# Autodesk Inventor assembly: populated-keyboard_cherrymx
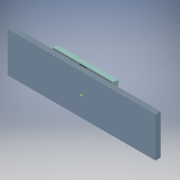
[picture p0: Inventor's stored thumbnail of the model, 180x180]
Saved by Autodesk Inventor 2018 (Build 220112000, 112)
## iProperties
Created: 2016-12-08
Part Number: populated-keyboard_cherrymx
Document SubType Name: Assembly
Designer: Cemra JC
Author: Cemra JC
## Documents named in this file (10)
- C:\Users\Jason Cemra\Documents\Logical Store\StenoToppers\stenotoppers\cherrymx\mockup-parts\populated-keyboard_cherrymx.iam
- C:\Users\Jason Cemra\Documents\Logical Store\StenoToppers\stenotoppers\cherrymx\mockup-parts\keyboard-mockup_cherrymx.iam
- C:\Users\Jason Cemra\Documents\Logical Store\StenoToppers\stenotoppers\cherrymx\mockup-parts\cherry-mx-switch\keyswitch_cherrymx.iam
- C:\Users\Jason Cemra\Documents\Logical Store\StenoToppers\stenotoppers\cherrymx\mockup-parts\spacebar-keycap_mockup_cherrymx.ipt
- C:\Users\Jason Cemra\Documents\Logical Store\StenoToppers\stenotoppers\cherrymx\stenotoppers\standard_cmx.ipt
- C:\Users\Jason Cemra\Documents\Logical Store\StenoToppers\stenotoppers\cherrymx\stenotoppers\smaller_cmx.ipt
- C:\Users\Jason Cemra\Documents\Logical Store\StenoToppers\stenotoppers\cherrymx\stenotoppers\larger_cmx.ipt
- C:\Users\Jason Cemra\Documents\Logical Store\StenoToppers\stenotoppers\cherrymx\stenotoppers\thumb_cmx.ipt
- J:\The Files\The Software Files\Projects\stenotoppers\cherrymx\stenotoppers.ipt
- C:\Users\Jason Cemra\Documents\Logical Store\StenoToppers\stenotoppers\parameters.xlsx
## Components (29 placed, 9 different names)
1. keyboard-mockup_cherrymx:1 [sub-assembly] — Spacebar Switch Attachment, Rigid:11, Rigid:12, Rigid:13, Rigid:14, Rigid:15, Rigid:16, Rigid:17, Rigid:18
2. Larger Left — Rigid:12
3. Smaller Right — Rigid:16
4. Smaller Left — Rigid:13
5. Larger Right — Rigid:15
6. spacebar-keyswitch [sub-assembly] — Spacebar Switch Attachment, Spacebar Attachment
7. spacebar-keycap_mockup_cherrymx:1 — Spacebar Attachment
8. standard_cmx:1 — Rigid:11
9. standard_cmx:9
10. standard_cmx:10
11. standard_cmx:11
12. standard_cmx:12
13. standard_cmx:13
14. standard_cmx:14
15. standard_cmx:15
16. standard_cmx:16
17. standard_cmx:2 — Rigid:14
18. standard_cmx:18
19. standard_cmx:19
20. standard_cmx:20
21. standard_cmx:21
22. standard_cmx:22
23. standard_cmx:23
24. standard_cmx:24
25. standard_cmx:25
26. thumb_cmx:7
27. thumb_cmx:26 — Rigid:18
28. thumb_cmx:8 — Rigid:17
29. thumb_cmx:27
## Component patterns: Top Row (9 elements), Middle Row (9 elements), Thumbs Left (2 elements), Thumbs Right (2 elements)
## Relationships (10: WeldJoint 10)
- Spacebar Switch Attachment [WeldJoint]: keyboard-mockup_cherrymx:1 ↔ spacebar-keyswitch
- Spacebar Attachment [WeldJoint]: spacebar-keyswitch ↔ spacebar-keycap_mockup_cherrymx:1
- Rigid:11 [WeldJoint] (0.4 mm): keyboard-mockup_cherrymx:1 ↔ standard_cmx:1
- Rigid:12 [WeldJoint] (0.4 mm): keyboard-mockup_cherrymx:1 ↔ Larger Left
- Rigid:13 [WeldJoint] (0.4 mm): keyboard-mockup_cherrymx:1 ↔ Smaller Left
- Rigid:14 [WeldJoint] (0.4 mm): keyboard-mockup_cherrymx:1 ↔ standard_cmx:2
- Rigid:15 [WeldJoint] (0.4 mm): keyboard-mockup_cherrymx:1 ↔ Larger Right
- Rigid:16 [WeldJoint] (0.4 mm): keyboard-mockup_cherrymx:1 ↔ Smaller Right
- Rigid:17 [WeldJoint] (0.4 mm): keyboard-mockup_cherrymx:1 ↔ thumb_cmx:8
- Rigid:18 [WeldJoint] (0.4 mm): keyboard-mockup_cherrymx:1 ↔ thumb_cmx:26
## Named parameters: k_width = 18 mm, k_height = 16.5 mm, k_height_t = 16 mm, k_taper1 = 1.5 mm, k_taper2 = 0.5 mm, k_staper = 1 mm, k_sradius = 4 mm, k_ltaper = 1.5 mm, k_lradius = 6 mm, k_radius = 6 mm, k_wthick = 1.5 mm, k_ribthick = 1.5 mm, k_ribheight = 5 mm, k_poleoff = 2.25 mm, k_poledia = 5.3 mm, k_cmxw = 1.1 mm, k_cmxl = 4.15 mm, s_bwidth = 14.4 mm, s_poleh = 3.6 mm, s_polebw = 5.4 mm, s_polebl = 7.45 mm, b_pad = 1 mm, b_tab = 27 mm, b_caps = 31.5 mm, b_lshift = 40.5 mm, b_rshift = 49.5 mm, b_ctrl = 22.5 mm, b_space = 117 mm, b_width = 285 mm, b_height = 77 mm, k_taper_thin = 0.0001 mm, k_height_low = 15 mm, k_taper_wide = 1.5 mm, k_shortening = 4.5 mm, k_cmxd = 4 mm, capgap = 0.4 mm, k_taper_side = 0.5 mm
